# Autodesk Inventor assembly: SMC_CJ2B16-175
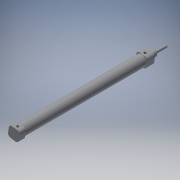
[picture p0: Inventor's stored thumbnail of the model, 180x180]
Saved by Autodesk Inventor 2018 (Build 220112000, 112)
## iProperties
Created: 2018-04-28
Part Number: SMC_CJ2B16-175
Material: 一般
Document SubType Name: Assembly
Designer: Take
Author: Take
## Documents named in this file (3)
- C:\Users\Take\Documents\Inventor\パーツ\SMC_CJ2B16-175.iam
- C:\Users\Take\Documents\Inventor\パーツ\SMC_CJ2B16-175(本体).ipt
- C:\Users\Take\Documents\Inventor\パーツ\SMC_CJ2B16-175(円柱).ipt
## Components (2 placed, 2 different names)
1. SMC_CJ2B16-175(本体):1 — 円柱状:1
2. SMC_CJ2B16-175(円柱):1 — 円柱状:1
## Relationships (1: CylindricalJoint 1)
- 円柱状:1 [CylindricalJoint]: SMC_CJ2B16-175(本体):1 ↔ SMC_CJ2B16-175(円柱):1
